# Autodesk Inventor assembly: TempLoggerRev1
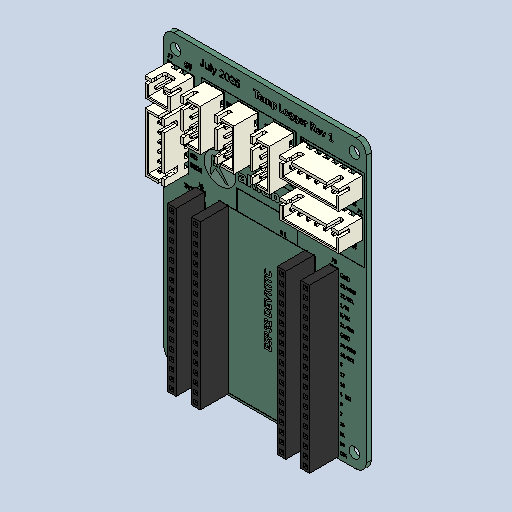
[picture p0: Inventor's stored thumbnail of the model, 512x512]
Saved by Autodesk Inventor 2026 (Build 300175050, 175E)
## iProperties
Company: Kicad
Created: 2025-07-16
Part Number: TempLoggerRev1
Description: KiCad electronic assembly
Document SubType Name: Assembly
Designer: kuzmin
Authority: Unknown
Sending System: KiCad to STEP converter
Preprocessor: Open CASCADE STEP processor 7.8
Title: TempLoggerRev1.step
Author: Pcbnew
## Documents named in this file (7)
- C:\Users\queez\Dropbox\Drawings\PIHTI\ElectronicsBox\esp32-ambient-logger\TempLoggerRev1.iam
- C:\Users\queez\Dropbox\Drawings\PIHTI\ElectronicsBox\esp32-ambient-logger\TempLoggerRev1\JST_XH_B4B-XH-A_1x04_P2.50mm_Vertical.ipt
- C:\Users\queez\Dropbox\Drawings\PIHTI\ElectronicsBox\esp32-ambient-logger\TempLoggerRev1\PinSocket_1x19_P2.54mm_Vertical.ipt
- C:\Users\queez\Dropbox\Drawings\PIHTI\ElectronicsBox\esp32-ambient-logger\TempLoggerRev1\JST_XH_B6B-XH-A_1x06_P2.50mm_Vertical.ipt
- C:\Users\queez\Dropbox\Drawings\PIHTI\ElectronicsBox\esp32-ambient-logger\TempLoggerRev1\JST_XH_B2B-XH-A_1x02_P2.50mm_Vertical.ipt
- C:\Users\queez\Dropbox\Drawings\PIHTI\ElectronicsBox\esp32-ambient-logger\TempLoggerRev1\esp32breakout_silkscreen.ipt
- C:\Users\queez\Dropbox\Drawings\PIHTI\ElectronicsBox\esp32-ambient-logger\TempLoggerRev1\esp32breakout_PCB.ipt
## Components (13 placed, 12 different names)
1. 1
2. 2 — Flush:2, Mate:3
3. 3
4. 4
5. 5 — Flush:1, Mate:4
6. 6
7. 7
8. 8
9. 9
10. 10
11. 11 — Mate:1, Mate:2
12. PinSocket_1x19_P2.54mm_Vertical:3 — Flush:2, Mate:2, Mate:3
13. PinSocket_1x19_P2.54mm_Vertical:4 — Flush:1, Mate:1, Mate:4
## Relationships (6: Mate 4, Flush 2)
- Flush:1: 5 ↔ PinSocket_1x19_P2.54mm_Vertical:4
- Flush:2: 2 ↔ PinSocket_1x19_P2.54mm_Vertical:3
- Mate:1: 11 ↔ PinSocket_1x19_P2.54mm_Vertical:4
- Mate:2: 11 ↔ PinSocket_1x19_P2.54mm_Vertical:3
- Mate:3 (4.55 mm): 2 ↔ PinSocket_1x19_P2.54mm_Vertical:3
- Mate:4 (4.5 mm): 5 ↔ PinSocket_1x19_P2.54mm_Vertical:4
